# Autodesk Inventor assembly: EIXOS_X_Z
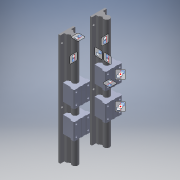
[picture p0: Inventor's stored thumbnail of the model, 180x180]
Saved by Autodesk Inventor 2018 (Build 220112000, 112)
## iProperties
Created: 2018-10-09
Part Number: EIXOS_X_Z
Material: Genérico
Document SubType Name: Assembly
Designer: Georgines
Author: Georgines
## Documents named in this file (3)
- C:\Users\Usuario\Documents\OpenCNC\MONTAGEM\CNC1\EIXOS_X_Z.iam
- C:\Users\Usuario\Documents\OpenCNC\COMPONENTES_MECANICOS\GUIAS_LINEARES\SBR16.ipt
- C:\Users\Usuario\Documents\OpenCNC\COMPONENTES_MECANICOS\BLOCOS_GUIAS_LINEARES\SBR16UU.ipt
## Components (8 placed, 2 different names)
1. SBR16:3 — Alinhamento:1, Coincidência:3, Alinhamento:5
2. SBR16:4 — Alinhamento:3, Coincidência:1, Alinhamento:8
3. SBR16:5 — Alinhamento:1, Coincidência:3, Alinhamento:5, Coincidência:6, Coincidência:7, Alinhamento:13, Coincidência:9, Alinhamento:14
4. SBR16:6 — Alinhamento:3, Coincidência:1, Alinhamento:8, Coincidência:5, Alinhamento:13, Coincidência:8, Coincidência:9, Alinhamento:14
5. SBR16UU:1 — Coincidência:5, Alinhamento:11, Alinhamento:12
6. SBR16UU:2 — Alinhamento:9, Alinhamento:10, Coincidência:8
7. SBR16UU:3 — Coincidência:6, Alinhamento:9, Alinhamento:10, Coincidência:10
8. SBR16UU:4 — Coincidência:7, Alinhamento:11, Alinhamento:12, Coincidência:10
## Relationships (18: Flush 10, Mate 8)
- Alinhamento:1 [Flush]: SBR16:3 ↔ SBR16:5
- Alinhamento:3 [Flush]: SBR16:4 ↔ SBR16:6
- Coincidência:1 [Mate]: SBR16:4 ↔ SBR16:6
- Coincidência:3 [Mate]: SBR16:3 ↔ SBR16:5
- Alinhamento:5 [Flush]: SBR16:3 ↔ SBR16:5
- Alinhamento:8 [Flush]: SBR16:4 ↔ SBR16:6
- Coincidência:5 [Mate]: SBR16:6 ↔ SBR16UU:1
- Coincidência:6 [Mate]: SBR16:5 ↔ SBR16UU:3
- Coincidência:7 [Mate]: SBR16:5 ↔ SBR16UU:4
- Alinhamento:9 [Flush]: SBR16UU:2 ↔ SBR16UU:3
- Alinhamento:10 [Flush]: SBR16UU:2 ↔ SBR16UU:3
- Alinhamento:11 [Flush]: SBR16UU:1 ↔ SBR16UU:4
- Alinhamento:12 [Flush]: SBR16UU:1 ↔ SBR16UU:4
- Alinhamento:13 [Flush]: SBR16:5 ↔ SBR16:6
- Coincidência:8 [Mate]: SBR16:6 ↔ SBR16UU:2
- Coincidência:9 [Mate] (45 mm): SBR16:5 ↔ SBR16:6
- Alinhamento:14 [Flush]: SBR16:5 ↔ SBR16:6
- Coincidência:10 [Mate] (30 mm): SBR16UU:3 ↔ SBR16UU:4
